# Autodesk Inventor assembly: assist_wheel
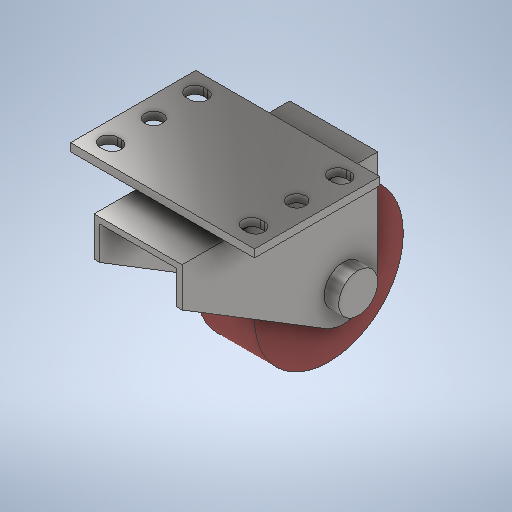
[picture p0: Inventor's stored thumbnail of the model, 512x512]
Saved by Autodesk Inventor 2026.2 (Build 302298010, 298A)
## iProperties
Created: 2026-03-29
Part Number: assist_wheel
Document SubType Name: Assembly
Designer: chanh
Author: chanh
## Documents named in this file (3)
- C:\Users\chanh\내 드라이브\교과공부\2026년 1학기 (4학년 1학기)\01창의제품설계\CLOSE_hardware\02하체\assist_wheel.iam
- C:\Users\chanh\내 드라이브\교과공부\2026년 1학기 (4학년 1학기)\01창의제품설계\CLOSE_hardware\02하체\assist_wheel.ipt
- C:\Users\chanh\내 드라이브\교과공부\2026년 1학기 (4학년 1학기)\01창의제품설계\CLOSE_hardware\02하체\assist_wheel_upper.ipt
## Components (2 placed, 2 different names)
1. assist_wheel:1 — Flush:1, Flush:2, Flush:3, Rotational:1
2. assist_wheel_upper:1 — Rotational:1
## Relationships (4: Flush 3, RevoluteJoint 1)
- Flush:1: assist_wheel:1
- Flush:2: assist_wheel:1
- Flush:3: assist_wheel:1
- Rotational:1 [RevoluteJoint]: assist_wheel:1 ↔ assist_wheel_upper:1
